# Autodesk Inventor assembly: 000-odom-v1
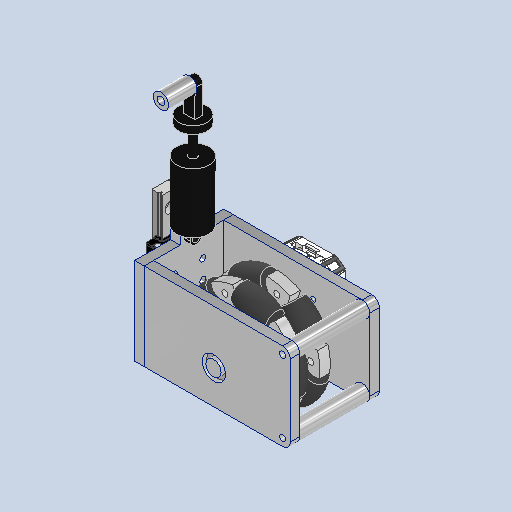
[picture p0: Inventor's stored thumbnail of the model, 512x512]
Saved by Autodesk Inventor 2025.2 (Build 292293000, 293)
## iProperties
Created: 2025-03-30
Part Number: 000-odom-v1
Document SubType Name: Assembly
Designer: haruy
Author: haruy
## Documents named in this file (13)
- C:\Users\haruy\Documents\ロボコン\NHK2025\cad\nagahisa\odom\000-odom-v1.iam
- C:\Users\haruy\Documents\ロボコン\NHK2025\cad\nagahisa\odom\SSEB-MX10-55.iam
- C:\Users\haruy\Documents\ロボコン\NHK2025\cad\nagahisa\odom\odom_v1_Plate_2.ipt
- C:\Users\haruy\Documents\ロボコン\NHK2025\cad\nagahisa\odom\odom_v1_Plate_3.ipt
- C:\Users\haruy\Documents\ロボコン\NHK2025\cad\nagahisa\odom\odom_v1_Plate_4.ipt
- C:\Users\haruy\Documents\ロボコン\NHK2025\cad\nagahisa\odom\bear_f8_12_sa.ipt
- C:\Users\haruy\Documents\ロボコン\NHK2025\cad\nagahisa\odom\odom_v1_shaft_1.ipt
- C:\Users\haruy\Documents\ロボコン\NHK2025\cad\000_parts\サスペンション\black-suspension.iam
- C:\Users\haruy\Documents\ロボコン\NHK2025\cad\nagahisa\odom\odom_v1_shaft_3.ipt
- C:\Users\haruy\Documents\ロボコン\NHK2025\cad\nagahisa\odom\amt102-v.iam
- C:\Users\haruy\Documents\ロボコン\NHK2025\cad\nagahisa\odom\odom_v1_shaft_4.ipt
- C:\Users\haruy\Documents\ロボコン\NHK2025\cad\nagahisa\odom\omni-60.ipt
- C:\Users\haruy\Documents\ロボコン\NHK2025\cad\nagahisa\odom\install-encoder-v1-3DP-Shaft-F.ipt
## Components (14 placed, 12 different names)
1. SSEB-MX10-55:1 [sub-assembly] — 挿入:3, 挿入:4
2. odom_v1_Plate_2:1 — 挿入:3, 挿入:4, 挿入:5, 挿入:6, 挿入:7, 挿入:8, 挿入:21
3. odom_v1_Plate_3:1 — 挿入:6, 挿入:8, 挿入:10, 挿入:17
4. odom_v1_Plate_4:1 — 挿入:5, 挿入:7, 挿入:9, 挿入:11, 挿入:12
5. bear_f8_12_sa:1 — 挿入:9, 挿入:18
6. bear_f8_12_sa:2 — 挿入:10
7. odom_v1_shaft_1:1 — 挿入:12
8. odom_v1_shaft_1:2 — 挿入:11
9. black-suspension:1 [sub-assembly] — 挿入:16, 挿入:21
10. odom_v1_shaft_3:1 — 挿入:16
11. amt102-v:1 [sub-assembly] — 挿入:17
12. odom_v1_shaft_4:1 — 挿入:18, 挿入:19
13. omni-60:1 — 挿入:19, 挿入:20
14. install-encoder-v1-3DP-Shaft-F:1 — 挿入:20
## Relationships (16: Insert 16)
- 挿入:3 [Insert]: SSEB-MX10-55:1 ↔ odom_v1_Plate_2:1
- 挿入:4 [Insert]: SSEB-MX10-55:1 ↔ odom_v1_Plate_2:1
- 挿入:5 [Insert]: odom_v1_Plate_2:1 ↔ odom_v1_Plate_4:1
- 挿入:6 [Insert]: odom_v1_Plate_2:1 ↔ odom_v1_Plate_3:1
- 挿入:7 [Insert]: odom_v1_Plate_2:1 ↔ odom_v1_Plate_4:1
- 挿入:8 [Insert]: odom_v1_Plate_2:1 ↔ odom_v1_Plate_3:1
- 挿入:9 [Insert]: odom_v1_Plate_4:1 ↔ bear_f8_12_sa:1
- 挿入:10 [Insert]: odom_v1_Plate_3:1 ↔ bear_f8_12_sa:2
- 挿入:11 [Insert]: odom_v1_Plate_4:1 ↔ odom_v1_shaft_1:2
- 挿入:12 [Insert]: odom_v1_Plate_4:1 ↔ odom_v1_shaft_1:1
- 挿入:16 [Insert]: black-suspension:1 ↔ odom_v1_shaft_3:1
- 挿入:17 [Insert]: odom_v1_Plate_3:1 ↔ amt102-v:1
- 挿入:18 [Insert]: bear_f8_12_sa:1 ↔ odom_v1_shaft_4:1
- 挿入:19 [Insert] (8.7 mm): odom_v1_shaft_4:1 ↔ omni-60:1
- 挿入:20 [Insert]: omni-60:1 ↔ install-encoder-v1-3DP-Shaft-F:1
- 挿入:21 [Insert]: odom_v1_Plate_2:1 ↔ black-suspension:1
